# Autodesk Inventor assembly: Assembly_IM_Design_Insert
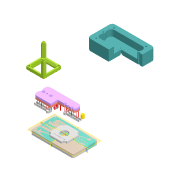
[picture p0: Inventor's stored thumbnail of the model, 180x180]
Saved by Autodesk Inventor 2022 (Build 260153000, 153)
## iProperties
Company: UNSPECIFIED
Created: 1900-01-01
Part Number: Assembly_IM_Design_Insert
Description: STEP AP203
Document SubType Name: Assembly
Designer: diederichbenedict
Sending System: ASCON Math Kernel
Preprocessor: ASCON STEP Converter 1.3
Title: assembly
Author: UNSPECIFIED
Revision Number: ANYUNSPECIFIED
## Documents named in this file (13)
- C:\Users\diederichbenedict\Dropbox\Dokumente\Promotion\PROJECTS\INJECTIONMOLDING\INVENTOR\Assembly_IM_Design_Insert.iam
- C:\Users\diederichbenedict\Dropbox\Dokumente\Promotion\PROJECTS\INJECTIONMOLDING\INVENTOR\Òåëî 1.iam
- C:\Users\diederichbenedict\Dropbox\Dokumente\Promotion\PROJECTS\INJECTIONMOLDING\INVENTOR\Òåëî 1_1.iam
- C:\Users\diederichbenedict\Dropbox\Dokumente\Promotion\PROJECTS\INJECTIONMOLDING\INVENTOR\Òåëî 1.ipt
- C:\Users\diederichbenedict\Dropbox\Dokumente\Promotion\PROJECTS\INJECTIONMOLDING\INVENTOR\Òåëî 1_1.ipt
- C:\Users\diederichbenedict\Dropbox\Dokumente\Promotion\PROJECTS\INJECTIONMOLDING\INVENTOR\Òåëî 1_2.ipt
- C:\Users\diederichbenedict\Dropbox\Dokumente\Promotion\PROJECTS\INJECTIONMOLDING\INVENTOR\Òåëî 1_3.ipt
- C:\Users\diederichbenedict\Dropbox\Dokumente\Promotion\PROJECTS\INJECTIONMOLDING\INVENTOR\Òåëî 1_4.ipt
- C:\Users\diederichbenedict\Dropbox\Dokumente\Promotion\PROJECTS\INJECTIONMOLDING\INVENTOR\Òåëî 1_5.ipt
- C:\Users\diederichbenedict\Dropbox\Dokumente\Promotion\PROJECTS\INJECTIONMOLDING\INVENTOR\Äåòàëü.ipt
- C:\Users\diederichbenedict\Dropbox\Dokumente\Promotion\PROJECTS\INJECTIONMOLDING\INVENTOR\10_Cube_base.ipt
- C:\Users\diederichbenedict\Dropbox\Dokumente\Promotion\PROJECTS\INJECTIONMOLDING\INVENTOR\20_Cube_Insert_Template_v3.ipt
- C:\Users\diederichbenedict\Dropbox\Dokumente\Promotion\PROJECTS\INJECTIONMOLDING\INVENTOR\01_Mold_Base_CubeInsert_v0.ipt
## Components (38 placed, 38 different names)
1. 5 [sub-assembly] — Fluchtend:1, Fluchtend:2, Passend:2
2. 10 [sub-assembly]
3. 11
4. 12
5. 13
6. 14
7. 16
8. 17
9. 18
10. 19
11. 20
12. 21
13. 22
14. 24
15. 25
16. 27
17. 28
18. 29
19. 30
20. 31
21. 32
22. 35
23. 36
24. 37
25. 38
26. 43
27. 44
28. 45
29. 46
30. 47
31. 48
32. 50
33. 51
34. 52
35. 53
36. 10_Cube_base:1
37. 20_Cube_Insert_Template_v3:1 — Fluchtend:3, Passend:1, Passend:2
38. 01_Mold_Base_CubeInsert_v0:1 — Fluchtend:1, Fluchtend:2, Fluchtend:3, Passend:1
## Relationships (5: Flush 3, Mate 2)
- Fluchtend:1 [Flush]: 5 ↔ 01_Mold_Base_CubeInsert_v0:1
- Fluchtend:2 [Flush]: 5 ↔ 01_Mold_Base_CubeInsert_v0:1
- Fluchtend:3 [Flush]: 20_Cube_Insert_Template_v3:1 ↔ 01_Mold_Base_CubeInsert_v0:1
- Passend:1 [Mate]: 20_Cube_Insert_Template_v3:1 ↔ 01_Mold_Base_CubeInsert_v0:1
- Passend:2 [Mate] (-5 mm): 5 ↔ 20_Cube_Insert_Template_v3:1
